# Autodesk Inventor assembly: ASSEMBLY_Main
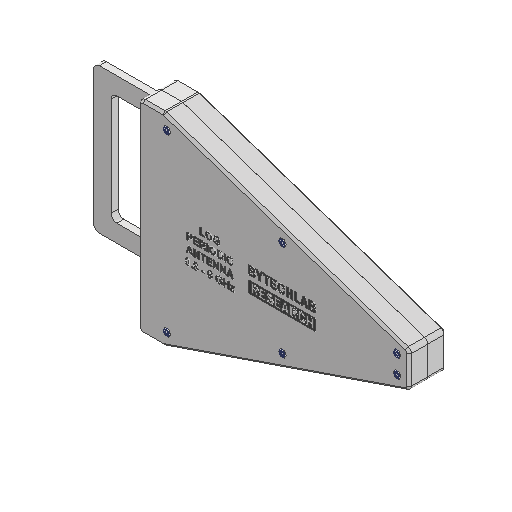
[picture p0: Inventor's stored thumbnail of the model, 512x512]
Saved by Autodesk Inventor 2026.1 (Build 301233000, 233)
## iProperties
Created: 2025-10-18
Part Number: ASSEMBLY_Main
Document SubType Name: Assembly
Designer: User
Author: User
## Documents named in this file (10)
- C:\Users\Andrzej\OneDrive\_DRIVE_SYNCH_FILES\RFC - #2 PCB Log Periodic Antenna (0.8-6 GHz)\MCAD\3_WITH_CASE_AND_FEED_COAX_FR4_V1\ASSEMBLY_MAIN_REVA\ASSEMBLY_Main.iam
- C:\Users\Andrzej\OneDrive\_DRIVE_SYNCH_FILES\RFC - #2 PCB Log Periodic Antenna (0.8-6 GHz)\MCAD\3_WITH_CASE_AND_FEED_COAX_FR4_V1\__KICAD_PCB_PARTS\ASSEMBLY_PCB_LOG_PERIODIC\ASSEMBLY_PCB_LOG_PERIODIC.iam
- C:\Users\Andrzej\OneDrive\_DRIVE_SYNCH_FILES\RFC - #2 PCB Log Periodic Antenna (0.8-6 GHz)\MCAD\3_WITH_CASE_AND_FEED_COAX_FR4_V1\__COTS_PARTS\COTS_GENERIC_RG316_COAX.ipt
- C:\Users\Andrzej\OneDrive\_DRIVE_SYNCH_FILES\RFC - #2 PCB Log Periodic Antenna (0.8-6 GHz)\MCAD\3_WITH_CASE_AND_FEED_COAX_FR4_V1\__COTS_PARTS\COTS_MOLEX_733910260_SMA_Connector\COTS_MOLEX_733910260_SMA_Connector.ipt
- C:\Users\Andrzej\OneDrive\_DRIVE_SYNCH_FILES\RFC - #2 PCB Log Periodic Antenna (0.8-6 GHz)\MCAD\3_WITH_CASE_AND_FEED_COAX_FR4_V1\ASSEMBLY_MAIN_REVA\3DP_PLA_Antenna_Case_Bottom.ipt
- C:\Users\Andrzej\OneDrive\_DRIVE_SYNCH_FILES\RFC - #2 PCB Log Periodic Antenna (0.8-6 GHz)\MCAD\3_WITH_CASE_AND_FEED_COAX_FR4_V1\__COTS_PARTS\COTS_DREMEC_8G205V50097_M3x30_Nylon_Screw.ipt
- C:\Users\Andrzej\OneDrive\_DRIVE_SYNCH_FILES\RFC - #2 PCB Log Periodic Antenna (0.8-6 GHz)\MCAD\3_WITH_CASE_AND_FEED_COAX_FR4_V1\__COTS_PARTS\COTS_BOSSARD_1400401_M3_Nylon_Nut.ipt
- C:\Users\Andrzej\OneDrive\_DRIVE_SYNCH_FILES\RFC - #2 PCB Log Periodic Antenna (0.8-6 GHz)\MCAD\3_WITH_CASE_AND_FEED_COAX_FR4_V1\ASSEMBLY_MAIN_REVA\3DP_PLA_Handle.ipt
- C:\Users\Andrzej\OneDrive\_DRIVE_SYNCH_FILES\RFC - #2 PCB Log Periodic Antenna (0.8-6 GHz)\MCAD\3_WITH_CASE_AND_FEED_COAX_FR4_V1\__COTS_PARTS\COTS_DREMEC_8G205M3X12_M3x12_Nylon_Screw.ipt
- C:\Users\Andrzej\OneDrive\_DRIVE_SYNCH_FILES\RFC - #2 PCB Log Periodic Antenna (0.8-6 GHz)\MCAD\3_WITH_CASE_AND_FEED_COAX_FR4_V1\ASSEMBLY_MAIN_REVA\ASSEMBLY_Antenna_Case_Top.iam
## Components (28 placed, 9 different names)
1. ASSEMBLY_PCB_LOG_PERIODIC:1 [sub-assembly] — Mate:1, Flush:1, Mate:2, Mate:5, Mate:6, Mate:7
2. COTS_GENERIC_RG316_COAX:1 — Mate:1, Flush:1, Mate:2, Mate:3, Mate:4
3. COTS_MOLEX_733910260_SMA_Connector:1 — Mate:3, Mate:4, Angle:12
4. 3DP_PLA_Antenna_Case_Bottom:1 — Mate:5, Mate:6, Mate:7, Mate:8, Flush:2, Flush:3, Mate:9, Mate:10, Mate:11, Mate:12, Mate:13, Mate:14, Mate:15, Mate:16, Mate:17, Mate:18, Mate:19, Mate:20, Mate:33, Mate:34, Mate:35, Mate:54, Mate:55, Mate:56, Mate:57, Mate:58, Angle:1, Angle:2, Angle:3, Angle:4, Angle:5, Angle:12
5. ASSEMBLY_Antenna_Case_Top:1 [sub-assembly] — Mate:8, Flush:2, Flush:3, Mate:27, Mate:28, Mate:29, Mate:30, Mate:31, Mate:32, Angle:6, Angle:7, Angle:8, Angle:9, Angle:10, Angle:11
6. COTS_DREMEC_8G205V50097_M3x30_Nylon_Screw:1 — Mate:9, Mate:20, Mate:22
7. COTS_DREMEC_8G205V50097_M3x30_Nylon_Screw:2 — Mate:10, Mate:18, Mate:23
8. COTS_DREMEC_8G205V50097_M3x30_Nylon_Screw:3 — Mate:11, Mate:16, Mate:24
9. COTS_DREMEC_8G205V50097_M3x30_Nylon_Screw:4 — Mate:12, Mate:19, Mate:21
10. COTS_DREMEC_8G205V50097_M3x30_Nylon_Screw:5 — Mate:13, Mate:17, Mate:26
11. COTS_DREMEC_8G205V50097_M3x30_Nylon_Screw:6 — Mate:14, Mate:15, Mate:25
12. COTS_BOSSARD_1400401_M3_Nylon_Nut:1 — Mate:25, Mate:27, Angle:11
13. COTS_BOSSARD_1400401_M3_Nylon_Nut:2 — Mate:26, Mate:31, Angle:10
14. COTS_BOSSARD_1400401_M3_Nylon_Nut:3 — Mate:22, Mate:30, Angle:8
15. COTS_BOSSARD_1400401_M3_Nylon_Nut:4 — Mate:24, Mate:28, Angle:6
16. COTS_BOSSARD_1400401_M3_Nylon_Nut:5 — Mate:21, Mate:32, Angle:9
17. COTS_BOSSARD_1400401_M3_Nylon_Nut:6 — Mate:23, Mate:29, Angle:7
18. 3DP_PLA_Handle:1 — Mate:33, Mate:34, Mate:35, Mate:36, Mate:37, Mate:38, Mate:39, Mate:40, Mate:41, Mate:48, Mate:49, Mate:50, Mate:51
19. COTS_DREMEC_8G205M3X12_M3x12_Nylon_Screw:1 — Mate:38, Mate:41, Mate:45
20. COTS_DREMEC_8G205M3X12_M3x12_Nylon_Screw:2 — Mate:37, Mate:40, Mate:46
21. COTS_DREMEC_8G205M3X12_M3x12_Nylon_Screw:3 — Mate:36, Mate:39, Mate:47
22. COTS_BOSSARD_1400401_M3_Nylon_Nut:7 — Mate:46, Mate:56, Angle:5
23. COTS_BOSSARD_1400401_M3_Nylon_Nut:8 — Mate:45, Mate:58, Angle:1
24. COTS_BOSSARD_1400401_M3_Nylon_Nut:9 — Mate:47, Mate:57, Angle:4
25. COTS_DREMEC_8G205M3X12_M3x12_Nylon_Screw:4 — Mate:49, Mate:51, Mate:53
26. COTS_DREMEC_8G205M3X12_M3x12_Nylon_Screw:5 — Mate:48, Mate:50, Mate:52
27. COTS_BOSSARD_1400401_M3_Nylon_Nut:10 — Mate:52, Mate:55, Angle:3
28. COTS_BOSSARD_1400401_M3_Nylon_Nut:11 — Mate:53, Mate:54, Angle:2
## Relationships (70: Mate 55, Angle 12, Flush 3)
- Mate:1: ASSEMBLY_PCB_LOG_PERIODIC:1 ↔ COTS_GENERIC_RG316_COAX:1
- Flush:1: ASSEMBLY_PCB_LOG_PERIODIC:1 ↔ COTS_GENERIC_RG316_COAX:1
- Mate:2: ASSEMBLY_PCB_LOG_PERIODIC:1 ↔ COTS_GENERIC_RG316_COAX:1
- Mate:3: COTS_GENERIC_RG316_COAX:1 ↔ COTS_MOLEX_733910260_SMA_Connector:1
- Mate:4: COTS_GENERIC_RG316_COAX:1 ↔ COTS_MOLEX_733910260_SMA_Connector:1
- Mate:5: ASSEMBLY_PCB_LOG_PERIODIC:1 ↔ 3DP_PLA_Antenna_Case_Bottom:1
- Mate:6: ASSEMBLY_PCB_LOG_PERIODIC:1 ↔ 3DP_PLA_Antenna_Case_Bottom:1
- Mate:7: ASSEMBLY_PCB_LOG_PERIODIC:1 ↔ 3DP_PLA_Antenna_Case_Bottom:1
- Mate:8: 3DP_PLA_Antenna_Case_Bottom:1 ↔ ASSEMBLY_Antenna_Case_Top:1
- Flush:2: 3DP_PLA_Antenna_Case_Bottom:1 ↔ ASSEMBLY_Antenna_Case_Top:1
- Flush:3: 3DP_PLA_Antenna_Case_Bottom:1 ↔ ASSEMBLY_Antenna_Case_Top:1
- Mate:9: 3DP_PLA_Antenna_Case_Bottom:1 ↔ COTS_DREMEC_8G205V50097_M3x30_Nylon_Screw:1
- Mate:10: 3DP_PLA_Antenna_Case_Bottom:1 ↔ COTS_DREMEC_8G205V50097_M3x30_Nylon_Screw:2
- Mate:11: 3DP_PLA_Antenna_Case_Bottom:1 ↔ COTS_DREMEC_8G205V50097_M3x30_Nylon_Screw:3
- Mate:12: 3DP_PLA_Antenna_Case_Bottom:1 ↔ COTS_DREMEC_8G205V50097_M3x30_Nylon_Screw:4
- Mate:13: 3DP_PLA_Antenna_Case_Bottom:1 ↔ COTS_DREMEC_8G205V50097_M3x30_Nylon_Screw:5
- Mate:14: 3DP_PLA_Antenna_Case_Bottom:1 ↔ COTS_DREMEC_8G205V50097_M3x30_Nylon_Screw:6
- Mate:15: 3DP_PLA_Antenna_Case_Bottom:1 ↔ COTS_DREMEC_8G205V50097_M3x30_Nylon_Screw:6
- Mate:16: 3DP_PLA_Antenna_Case_Bottom:1 ↔ COTS_DREMEC_8G205V50097_M3x30_Nylon_Screw:3
- Mate:17: 3DP_PLA_Antenna_Case_Bottom:1 ↔ COTS_DREMEC_8G205V50097_M3x30_Nylon_Screw:5
- Mate:18: 3DP_PLA_Antenna_Case_Bottom:1 ↔ COTS_DREMEC_8G205V50097_M3x30_Nylon_Screw:2
- Mate:19: 3DP_PLA_Antenna_Case_Bottom:1 ↔ COTS_DREMEC_8G205V50097_M3x30_Nylon_Screw:4
- Mate:20: 3DP_PLA_Antenna_Case_Bottom:1 ↔ COTS_DREMEC_8G205V50097_M3x30_Nylon_Screw:1
- Mate:21: COTS_DREMEC_8G205V50097_M3x30_Nylon_Screw:4 ↔ COTS_BOSSARD_1400401_M3_Nylon_Nut:5
- Mate:22: COTS_DREMEC_8G205V50097_M3x30_Nylon_Screw:1 ↔ COTS_BOSSARD_1400401_M3_Nylon_Nut:3
- Mate:23: COTS_DREMEC_8G205V50097_M3x30_Nylon_Screw:2 ↔ COTS_BOSSARD_1400401_M3_Nylon_Nut:6
- Mate:24: COTS_DREMEC_8G205V50097_M3x30_Nylon_Screw:3 ↔ COTS_BOSSARD_1400401_M3_Nylon_Nut:4
- Mate:25: COTS_DREMEC_8G205V50097_M3x30_Nylon_Screw:6 ↔ COTS_BOSSARD_1400401_M3_Nylon_Nut:1
- Mate:26: COTS_DREMEC_8G205V50097_M3x30_Nylon_Screw:5 ↔ COTS_BOSSARD_1400401_M3_Nylon_Nut:2
- Mate:27: ASSEMBLY_Antenna_Case_Top:1 ↔ COTS_BOSSARD_1400401_M3_Nylon_Nut:1
- Mate:28: ASSEMBLY_Antenna_Case_Top:1 ↔ COTS_BOSSARD_1400401_M3_Nylon_Nut:4
- Mate:29: ASSEMBLY_Antenna_Case_Top:1 ↔ COTS_BOSSARD_1400401_M3_Nylon_Nut:6
- Mate:30: ASSEMBLY_Antenna_Case_Top:1 ↔ COTS_BOSSARD_1400401_M3_Nylon_Nut:3
- Mate:31: ASSEMBLY_Antenna_Case_Top:1 ↔ COTS_BOSSARD_1400401_M3_Nylon_Nut:2
- Mate:32: ASSEMBLY_Antenna_Case_Top:1 ↔ COTS_BOSSARD_1400401_M3_Nylon_Nut:5
- Mate:33: 3DP_PLA_Antenna_Case_Bottom:1 ↔ 3DP_PLA_Handle:1
- Mate:34: 3DP_PLA_Antenna_Case_Bottom:1 ↔ 3DP_PLA_Handle:1
- Mate:35: 3DP_PLA_Antenna_Case_Bottom:1 ↔ 3DP_PLA_Handle:1
- Mate:36: 3DP_PLA_Handle:1 ↔ COTS_DREMEC_8G205M3X12_M3x12_Nylon_Screw:3
- Mate:37: 3DP_PLA_Handle:1 ↔ COTS_DREMEC_8G205M3X12_M3x12_Nylon_Screw:2
- Mate:38: 3DP_PLA_Handle:1 ↔ COTS_DREMEC_8G205M3X12_M3x12_Nylon_Screw:1
- Mate:39: 3DP_PLA_Handle:1 ↔ COTS_DREMEC_8G205M3X12_M3x12_Nylon_Screw:3
- Mate:40: 3DP_PLA_Handle:1 ↔ COTS_DREMEC_8G205M3X12_M3x12_Nylon_Screw:2
- Mate:41: 3DP_PLA_Handle:1 ↔ COTS_DREMEC_8G205M3X12_M3x12_Nylon_Screw:1
- Mate:45: COTS_DREMEC_8G205M3X12_M3x12_Nylon_Screw:1 ↔ COTS_BOSSARD_1400401_M3_Nylon_Nut:8
- Mate:46: COTS_DREMEC_8G205M3X12_M3x12_Nylon_Screw:2 ↔ COTS_BOSSARD_1400401_M3_Nylon_Nut:7
- Mate:47: COTS_DREMEC_8G205M3X12_M3x12_Nylon_Screw:3 ↔ COTS_BOSSARD_1400401_M3_Nylon_Nut:9
- Mate:48: 3DP_PLA_Handle:1 ↔ COTS_DREMEC_8G205M3X12_M3x12_Nylon_Screw:5
- Mate:49: 3DP_PLA_Handle:1 ↔ COTS_DREMEC_8G205M3X12_M3x12_Nylon_Screw:4
- Mate:50: 3DP_PLA_Handle:1 ↔ COTS_DREMEC_8G205M3X12_M3x12_Nylon_Screw:5
- Mate:51: 3DP_PLA_Handle:1 ↔ COTS_DREMEC_8G205M3X12_M3x12_Nylon_Screw:4
- Mate:52: COTS_DREMEC_8G205M3X12_M3x12_Nylon_Screw:5 ↔ COTS_BOSSARD_1400401_M3_Nylon_Nut:10
- Mate:53: COTS_DREMEC_8G205M3X12_M3x12_Nylon_Screw:4 ↔ COTS_BOSSARD_1400401_M3_Nylon_Nut:11
- Mate:54: 3DP_PLA_Antenna_Case_Bottom:1 ↔ COTS_BOSSARD_1400401_M3_Nylon_Nut:11
- Mate:55: 3DP_PLA_Antenna_Case_Bottom:1 ↔ COTS_BOSSARD_1400401_M3_Nylon_Nut:10
- Mate:56: 3DP_PLA_Antenna_Case_Bottom:1 ↔ COTS_BOSSARD_1400401_M3_Nylon_Nut:7
- Mate:57: 3DP_PLA_Antenna_Case_Bottom:1 ↔ COTS_BOSSARD_1400401_M3_Nylon_Nut:9
- Mate:58: 3DP_PLA_Antenna_Case_Bottom:1 ↔ COTS_BOSSARD_1400401_M3_Nylon_Nut:8
- Angle:1 (0 deg): 3DP_PLA_Antenna_Case_Bottom:1 ↔ COTS_BOSSARD_1400401_M3_Nylon_Nut:8
- Angle:2 (0 deg): 3DP_PLA_Antenna_Case_Bottom:1 ↔ COTS_BOSSARD_1400401_M3_Nylon_Nut:11
- Angle:3 (0 deg): 3DP_PLA_Antenna_Case_Bottom:1 ↔ COTS_BOSSARD_1400401_M3_Nylon_Nut:10
- Angle:4 (0 deg): 3DP_PLA_Antenna_Case_Bottom:1 ↔ COTS_BOSSARD_1400401_M3_Nylon_Nut:9
- Angle:5 (0 deg): 3DP_PLA_Antenna_Case_Bottom:1 ↔ COTS_BOSSARD_1400401_M3_Nylon_Nut:7
- Angle:6 (0 deg): ASSEMBLY_Antenna_Case_Top:1 ↔ COTS_BOSSARD_1400401_M3_Nylon_Nut:4
- Angle:7 (0 deg): ASSEMBLY_Antenna_Case_Top:1 ↔ COTS_BOSSARD_1400401_M3_Nylon_Nut:6
- Angle:8 (0 deg): ASSEMBLY_Antenna_Case_Top:1 ↔ COTS_BOSSARD_1400401_M3_Nylon_Nut:3
- Angle:9 (0 deg): ASSEMBLY_Antenna_Case_Top:1 ↔ COTS_BOSSARD_1400401_M3_Nylon_Nut:5
- Angle:10 (0 deg): ASSEMBLY_Antenna_Case_Top:1 ↔ COTS_BOSSARD_1400401_M3_Nylon_Nut:2
- Angle:11 (0 deg): ASSEMBLY_Antenna_Case_Top:1 ↔ COTS_BOSSARD_1400401_M3_Nylon_Nut:1
- Angle:12 (0 deg): COTS_MOLEX_733910260_SMA_Connector:1 ↔ 3DP_PLA_Antenna_Case_Bottom:1
